# Autodesk Inventor assembly: 組合檔
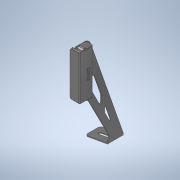
[picture p0: Inventor's stored thumbnail of the model, 180x180]
Saved by Autodesk Inventor 2020 (Build 240168000, 168)
## iProperties
Created: 2015-11-28
Part Number: 組合檔
Document SubType Name: Assembly
Designer: 設計製圖
Author: 設計製圖
## Documents named in this file (16)
- D:\資料庫\設計-3D Project\【May club 】\得利卡-車頂燈架\模型、圖面\版本-吊架-長(#11.26)\長-車頂燈架-組合(#11.26).iam
- D:\資料庫\設計-3D Project\【 鐵蹄 】\------鐵蹄工廠素材------ -\拉帽-M8.ipt
- D:\資料庫\設計-3D Project\【May club 】\得利卡-車頂燈架\模型、圖面\焊接組件-1(#11.02).ipt
- D:\資料庫\設計-3D Project\材料庫\【螺絲】\止付螺絲\止付螺絲-M8-20.ipt
- D:\資料庫\設計-3D Project\【May club 】\得利卡-車頂燈架\模型、圖面\車身圖.ipt
- D:\資料庫\設計-3D Project\【May club 】\得利卡-車頂燈架\模型、圖面\吊架組件-ㄇ槽(#11.02).ipt
- D:\資料庫\設計-3D Project\【May club 】\得利卡-車頂燈架\模型、圖面\焊接組件-2(#11.02).ipt
- D:\資料庫\設計-3D Project\材料庫\螺帽\白鐵-六角螺帽-M6.ipt
- D:\資料庫\設計-3D Project\【May club 】\得利卡-車頂燈架\模型、圖面\版本-吊架-長(#11.26)\概-泡棉墊2.5t(1).ipt
- D:\資料庫\設計-3D Project\【May club 】\得利卡-車頂燈架\模型、圖面\版本-吊架-長(#11.26)\概-泡棉墊6.0t(2).ipt
- D:\資料庫\設計-3D Project\【May club 】\得利卡-車頂燈架\模型、圖面\版本-吊架-長(#11.26)\吊架-長(R)(#11.26).ipt
- D:\資料庫\設計-3D Project\【May club 】\得利卡-車頂燈架\模型、圖面\版本-吊架-長(#11.26)\焊接組件-3(R)  ( #11.26).ipt
- D:\資料庫\設計-3D Project\材料庫\【螺絲】\外六角螺絲\白鐵-外六角  M6-20.ipt
- D:\資料庫\設計-3D Project\材料庫\【華司】\彈簧華司\白鐵-彈簧華司-6.ipt
- D:\資料庫\設計-3D Project\材料庫\【華司】\白鐵-平面華司-7-16-2t.ipt
- D:\資料庫\設計-3D Project\【May club 】\得利卡-車頂燈架\模型、圖面\得利卡-車頂導水槽.ipt
## Components (17 placed, 15 different names)
1. 得利卡-車頂導水槽:1 — 角度:1
2. 車身圖:1 — 貼合:33
3. 吊架-長(R)(#11.26):1 — 貼合:18, 貼合:23, 貼合:25, 貼合:26, 貼合:33, 齊平:18, 貼合:47, 齊平:19, 貼合:48, 貼合:54
4. 吊架組件-ㄇ槽(#11.02):1 — 貼合:6, 齊平:2, 齊平:3, 貼合:17, 貼合:37, 貼合:38, 貼合:40, 齊平:14, 貼合:41, 貼合:18, 齊平:13, 齊平:16, 角度:1
5. 焊接組件-1(#11.02):1 — 貼合:23, 貼合:25, 貼合:26, 貼合:27, 齊平:7, 齊平:8, 齊平:13, 齊平:16
6. 拉帽-M8:1 — 齊平:6, 貼合:15, 貼合:17, 貼合:31, 貼合:37, 齊平:20
7. 拉帽-M8:2 — 齊平:6, 貼合:15, 貼合:32, 貼合:38
8. 焊接組件-2(#11.02):1 — 貼合:40, 齊平:14, 貼合:41, 貼合:44, 貼合:45, 齊平:15
9. 白鐵-外六角  M6-20:1 — 貼合:46, 貼合:50, 貼合:51, 貼合:53
10. 白鐵-六角螺帽-M6:1 — 貼合:44, 貼合:45, 齊平:15, 貼合:46
11. 焊接組件-3(R)  ( #11.26):1 — 貼合:47, 齊平:19, 貼合:48
12. 白鐵-彈簧華司-6:1 — 貼合:50, 貼合:52, 貼合:53
13. 白鐵-平面華司-7-16-2t:1 — 貼合:51, 貼合:52, 貼合:54
14. 概-泡棉墊6.0t(2):1 — 貼合:27, 齊平:7, 齊平:8
15. 概-泡棉墊2.5t(1):1 — 貼合:6, 齊平:2, 齊平:3
16. 止付螺絲-M8-20:1 — 齊平:12, 貼合:31, 齊平:20
17. 止付螺絲-M8-20:2 — 齊平:12, 貼合:32
## Relationships (39: Mate 25, Flush 13, Angle 1)
- 貼合:6 [Mate]: 吊架組件-ㄇ槽(#11.02):1 ↔ 概-泡棉墊2.5t(1):1
- 齊平:2 [Flush]: 吊架組件-ㄇ槽(#11.02):1 ↔ 概-泡棉墊2.5t(1):1
- 齊平:3 [Flush]: 吊架組件-ㄇ槽(#11.02):1 ↔ 概-泡棉墊2.5t(1):1
- 齊平:6 [Flush]: 拉帽-M8:1 ↔ 拉帽-M8:2
- 貼合:15 [Mate]: 拉帽-M8:1 ↔ 拉帽-M8:2
- 貼合:17 [Mate]: 吊架組件-ㄇ槽(#11.02):1 ↔ 拉帽-M8:1
- 貼合:23 [Mate]: 吊架-長(R)(#11.26):1 ↔ 焊接組件-1(#11.02):1
- 貼合:25 [Mate]: 吊架-長(R)(#11.26):1 ↔ 焊接組件-1(#11.02):1
- 貼合:26 [Mate]: 吊架-長(R)(#11.26):1 ↔ 焊接組件-1(#11.02):1
- 貼合:27 [Mate]: 焊接組件-1(#11.02):1 ↔ 概-泡棉墊6.0t(2):1
- 齊平:7 [Flush]: 焊接組件-1(#11.02):1 ↔ 概-泡棉墊6.0t(2):1
- 齊平:8 [Flush]: 焊接組件-1(#11.02):1 ↔ 概-泡棉墊6.0t(2):1
- 齊平:12 [Flush]: 止付螺絲-M8-20:1 ↔ 止付螺絲-M8-20:2
- 貼合:31 [Mate]: 拉帽-M8:1 ↔ 止付螺絲-M8-20:1
- 貼合:32 [Mate]: 拉帽-M8:2 ↔ 止付螺絲-M8-20:2
- 貼合:33 [Mate]: 車身圖:1 ↔ 吊架-長(R)(#11.26):1
- 貼合:37 [Mate]: 吊架組件-ㄇ槽(#11.02):1 ↔ 拉帽-M8:1
- 貼合:38 [Mate]: 吊架組件-ㄇ槽(#11.02):1 ↔ 拉帽-M8:2
- 貼合:40 [Mate]: 吊架組件-ㄇ槽(#11.02):1 ↔ 焊接組件-2(#11.02):1
- 齊平:14 [Flush]: 吊架組件-ㄇ槽(#11.02):1 ↔ 焊接組件-2(#11.02):1
- 貼合:41 [Mate]: 吊架組件-ㄇ槽(#11.02):1 ↔ 焊接組件-2(#11.02):1
- 貼合:18 [Mate]: 吊架-長(R)(#11.26):1 ↔ 吊架組件-ㄇ槽(#11.02):1
- 齊平:13 [Flush]: 吊架組件-ㄇ槽(#11.02):1 ↔ 焊接組件-1(#11.02):1
- 貼合:44 [Mate]: 焊接組件-2(#11.02):1 ↔ 白鐵-六角螺帽-M6:1
- 貼合:45 [Mate]: 焊接組件-2(#11.02):1 ↔ 白鐵-六角螺帽-M6:1
- 齊平:15 [Flush]: 焊接組件-2(#11.02):1 ↔ 白鐵-六角螺帽-M6:1
- 貼合:46 [Mate]: 白鐵-外六角  M6-20:1 ↔ 白鐵-六角螺帽-M6:1
- 齊平:16 [Flush]: 吊架組件-ㄇ槽(#11.02):1 ↔ 焊接組件-1(#11.02):1
- 齊平:18 [Flush] (150 mm): 吊架-長(R)(#11.26):1
- 貼合:47 [Mate]: 吊架-長(R)(#11.26):1 ↔ 焊接組件-3(R)  ( #11.26):1
- 齊平:19 [Flush] (5 mm): 吊架-長(R)(#11.26):1 ↔ 焊接組件-3(R)  ( #11.26):1
- 貼合:48 [Mate] (0.5 mm): 吊架-長(R)(#11.26):1 ↔ 焊接組件-3(R)  ( #11.26):1
- 齊平:20 [Flush]: 拉帽-M8:1 ↔ 止付螺絲-M8-20:1
- 貼合:50 [Mate]: 白鐵-外六角  M6-20:1 ↔ 白鐵-彈簧華司-6:1
- 貼合:51 [Mate]: 白鐵-外六角  M6-20:1 ↔ 白鐵-平面華司-7-16-2t:1
- 貼合:52 [Mate]: 白鐵-彈簧華司-6:1 ↔ 白鐵-平面華司-7-16-2t:1
- 貼合:53 [Mate]: 白鐵-外六角  M6-20:1 ↔ 白鐵-彈簧華司-6:1
- 貼合:54 [Mate]: 吊架-長(R)(#11.26):1 ↔ 白鐵-平面華司-7-16-2t:1
- 角度:1 [Angle] (0 deg): 得利卡-車頂導水槽:1 ↔ 吊架組件-ㄇ槽(#11.02):1
